# Autodesk Inventor assembly: ASY MSC Жабры
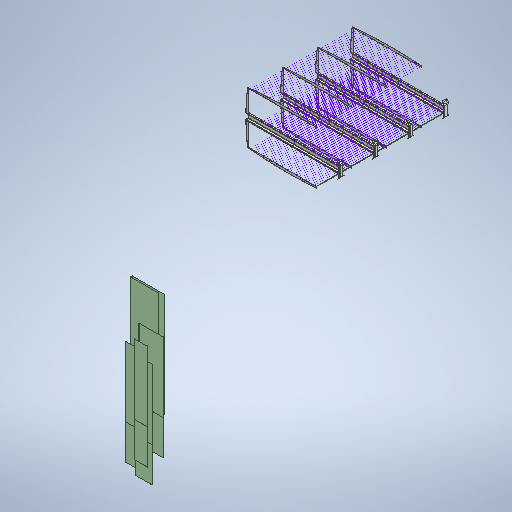
[picture p0: Inventor's stored thumbnail of the model, 512x512]
Saved by Autodesk Inventor 2025 (Build 290162010, 162A)
## iProperties
Created: 2024-08-31
Part Number: ASY MSC Жабры
Document SubType Name: Assembly
Designer: pokla
Author: pokla
## Documents named in this file (22)
- C:\Users\pokla\Documents\Inventor\Отстойник осветлитель\Manturovo_Se-clar-Gleb\ASY MSC Жабры.iam
- C:\Users\pokla\Documents\Inventor\Отстойник осветлитель\Manturovo_Se-clar-Gleb\MSC 0101 sheet gills.ipt
- C:\Users\pokla\Documents\Inventor\Отстойник осветлитель\Manturovo_Se-clar-Gleb\MSC 081 pillar 1.ipt
- C:\Users\pokla\Documents\Inventor\Отстойник осветлитель\Manturovo_Se-clar-Gleb\MSC 0102 sheet gills.ipt
- C:\Users\pokla\Documents\Inventor\Отстойник осветлитель\Manturovo_Se-clar-Gleb\MSC 0202 sheet gills.ipt
- C:\Users\pokla\Documents\Inventor\Отстойник осветлитель\Manturovo_Se-clar-Gleb\MSC 0103 sheet gills.ipt
- C:\Users\pokla\Documents\Inventor\Отстойник осветлитель\Manturovo_Se-clar-Gleb\MSC 0203 sheet gills.ipt
- C:\Users\pokla\Documents\Inventor\Отстойник осветлитель\Manturovo_Se-clar-Gleb\MSC 0104 sheet gills.ipt
- C:\Users\pokla\Documents\Inventor\Отстойник осветлитель\Manturovo_Se-clar-Gleb\MSC 0204 sheet gills.ipt
- C:\Users\pokla\Documents\Inventor\Отстойник осветлитель\Manturovo_Se-clar-Gleb\MSC 0105 sheet gills.ipt
- C:\Users\pokla\Documents\Inventor\Отстойник осветлитель\Manturovo_Se-clar-Gleb\MSC 0205 sheet gills.ipt
- C:\Users\pokla\Documents\Inventor\Отстойник осветлитель\Manturovo_Se-clar-Gleb\MSC 0106 sheet gills.ipt
- C:\Users\pokla\Documents\Inventor\Отстойник осветлитель\Manturovo_Se-clar-Gleb\MSC 0206 sheet gills.ipt
- C:\Users\pokla\Documents\Inventor\Отстойник осветлитель\Manturovo_Se-clar-Gleb\MSC 0107 sheet gills.ipt
- C:\Users\pokla\Documents\Inventor\Отстойник осветлитель\Manturovo_Se-clar-Gleb\MSC 0207 sheet gills.ipt
- C:\Users\pokla\Documents\Inventor\Отстойник осветлитель\Manturovo_Se-clar-Gleb\MSC 079 creen pillar.ipt
- C:\Users\pokla\Documents\Inventor\Отстойник осветлитель\Manturovo_Se-clar-Gleb\MSC DIM 085 tube belly.ipt
- C:\Users\pokla\Documents\Inventor\Отстойник осветлитель\Manturovo_Se-clar-Gleb\MSC 081 pillar 1_CPY.ipt
- C:\Users\pokla\Documents\Inventor\Отстойник осветлитель\Manturovo_Se-clar-Gleb\MSC 0211 string for sheets.ipt
- C:\Users\pokla\Documents\Inventor\Отстойник осветлитель\Manturovo_Se-clar-Gleb\MSC 079 top pillar.ipt
- C:\Users\pokla\Documents\Inventor\Отстойник осветлитель\Manturovo_Se-clar-Gleb\MSC DIM 085.1 heel.ipt
- C:\Users\pokla\Documents\Inventor\Отстойник осветлитель\Manturovo_Se-clar-Gleb\MSC 0201 sheet gills.ipt
## Components (184 placed, 21 different names)
1. MSC 0101 sheet gills.ipt:1 — Tangent:1, Tangent:2, Tangent:3, Flush:6, Flush:7, Flush:8, Mate:14
2. MSC 0201 sheet gills:1 — Flush:7, Flush:8, Mate:14
3. MSC 0102 sheet gills:1 — Rigid:17
4. MSC 0202 sheet gills:1 — Rigid:17
5. MSC 0103 sheet gills:1 — Rigid:18
6. MSC 0203 sheet gills:1 — Rigid:18
7. MSC 0104 sheet gills:1 — Rigid:19
8. MSC 0204 sheet gills:1 — Rigid:19
9. MSC 0105 sheet gills:1 — Rigid:20
10. MSC 0205 sheet gills:1 — Rigid:20
11. MSC 0106 sheet gills:1 — Rigid:21
12. MSC 0206 sheet gills:1 — Rigid:21
13. MSC 0107 sheet gills:1 — Rigid:22
14. MSC 0207 sheet gills:1 — Rigid:22
15. MSC 079 creen pillar:1 — Rigid:11, Rigid:12
16. MSC 081 pillar 1_CPY:1 — Rigid:8, Rigid:9
17. MSC 079 top pillar:1 — Rigid:8, Rigid:11
18. MSC 079 top pillar:2 — Rigid:9, Rigid:10
19. MSC 079 creen pillar:2 — Rigid:10, Rigid:15
20. MSC 081 pillar 1:1 — Mate:11, Mate:12, Mate:13, Rigid:13, Rigid:16, Flush:6
21. MSC DIM 085 tube belly:1 — Rigid:6, Rigid:7, Mate:11, Mate:12, Mate:13, Mate:15, Mate:16, Flush:9
22. MSC DIM 085.1 heel:1 — Rigid:7
23. MSC DIM 085.1 heel:2 — Rigid:6
24. MSC 079 creen pillar:3
25. MSC 081 pillar 1_CPY:2
26. MSC 079 top pillar:3
27. MSC 079 top pillar:4
28. MSC 079 creen pillar:4
29. MSC 081 pillar 1:2
30. MSC DIM 085 tube belly:2
31. MSC DIM 085.1 heel:3
32. MSC DIM 085.1 heel:4
33. MSC 079 creen pillar:5
34. MSC 081 pillar 1_CPY:3
35. MSC 079 top pillar:5
36. MSC 079 top pillar:6
37. MSC 079 creen pillar:6
38. MSC 081 pillar 1:3
39. MSC DIM 085 tube belly:3
40. MSC DIM 085.1 heel:5
41. MSC DIM 085.1 heel:6
42. MSC 079 creen pillar:7
43. MSC 081 pillar 1_CPY:4
44. MSC 079 top pillar:7
45. MSC 079 top pillar:8
46. MSC 079 creen pillar:8
47. MSC 081 pillar 1:4
48. MSC DIM 085 tube belly:4
49. MSC DIM 085.1 heel:7
50. MSC DIM 085.1 heel:8
51. MSC 0211 string for sheets:4 — Rigid:15
52. MSC 0211 string for sheets:2 — Rigid:12, Tangent:1, Tangent:2
53. MSC 0211 string for sheets:5
54. MSC 0211 string for sheets:6
55. MSC 0211 string for sheets:7
56. MSC 0211 string for sheets:8
57. MSC 0211 string for sheets:9
58. MSC 0211 string for sheets:10
59. MSC 0211 string for sheets:11
60. MSC 0211 string for sheets:12
61. MSC 0211 string for sheets:13
62. MSC 0211 string for sheets:14
63. MSC 0211 string for sheets:15
64. MSC 0211 string for sheets:16
65. MSC 0211 string for sheets:17
66. MSC 0211 string for sheets:18
67. MSC 0211 string for sheets:19
68. MSC 0211 string for sheets:20
69. MSC 0211 string for sheets:21
70. MSC 0211 string for sheets:22
71. MSC 0211 string for sheets:23
72. MSC 0211 string for sheets:24
73. MSC 0211 string for sheets:25
74. MSC 0211 string for sheets:26
75. MSC 0211 string for sheets:27
76. MSC 0211 string for sheets:28
77. MSC 0211 string for sheets:29
78. MSC 0211 string for sheets:30
79. MSC 0211 string for sheets:31
80. MSC 0211 string for sheets:32
81. MSC 0211 string for sheets:33
82. MSC 0211 string for sheets:34
83. MSC 0211 string for sheets:35
84. MSC 0211 string for sheets:36
85. MSC 0211 string for sheets:37
86. MSC 0211 string for sheets:38
87. MSC 0211 string for sheets:39
88. MSC 0211 string for sheets:40
89. MSC 0211 string for sheets:41
90. MSC 0211 string for sheets:42
91. MSC 0211 string for sheets:43
92. MSC 0211 string for sheets:44
93. MSC 0211 string for sheets:45
94. MSC 0211 string for sheets:46
95. MSC 0211 string for sheets:47
96. MSC 0211 string for sheets:48
97. MSC 0211 string for sheets:49
98. MSC 0211 string for sheets:50
99. MSC 0211 string for sheets:51
100. MSC 0211 string for sheets:52
101. MSC 0211 string for sheets:53
102. MSC 0211 string for sheets:54
103. MSC 0211 string for sheets:55
104. MSC 0211 string for sheets:56
105. MSC 0211 string for sheets:57
106. MSC 0211 string for sheets:58
107. MSC 0211 string for sheets:59
108. MSC 0211 string for sheets:60
109. MSC 0211 string for sheets:61
110. MSC 0211 string for sheets:62
111. MSC 0211 string for sheets:63
112. MSC 0211 string for sheets:64
113. MSC 0211 string for sheets:3 — Rigid:16
114. MSC 0211 string for sheets:1 — Rigid:13, Tangent:3
115. MSC 0211 string for sheets:65
116. MSC 0211 string for sheets:66
117. MSC 0211 string for sheets:67
118. MSC 0211 string for sheets:68
119. MSC 0211 string for sheets:69
120. MSC 0211 string for sheets:70
121. MSC 0211 string for sheets:71
122. MSC 0211 string for sheets:72
123. MSC 0211 string for sheets:73
124. MSC 0211 string for sheets:74
125. MSC 0211 string for sheets:75
126. MSC 0211 string for sheets:76
127. MSC 0211 string for sheets:77
128. MSC 0211 string for sheets:78
129. MSC 0211 string for sheets:79
130. MSC 0211 string for sheets:80
131. MSC 0211 string for sheets:81
132. MSC 0211 string for sheets:82
133. MSC 0211 string for sheets:83
134. MSC 0211 string for sheets:84
135. MSC 0211 string for sheets:85
136. MSC 0211 string for sheets:86
137. MSC 0211 string for sheets:87
138. MSC 0211 string for sheets:88
139. MSC 0211 string for sheets:89
140. MSC 0211 string for sheets:90
141. MSC 0211 string for sheets:91
142. MSC 0211 string for sheets:92
143. MSC 0211 string for sheets:93
144. MSC 0211 string for sheets:94
145. MSC 0211 string for sheets:95
146. MSC 0211 string for sheets:96
147. MSC 0211 string for sheets:97
148. MSC 0211 string for sheets:98
149. MSC 0211 string for sheets:99
150. MSC 0211 string for sheets:100
151. MSC 0211 string for sheets:101
152. MSC 0211 string for sheets:102
153. MSC 0211 string for sheets:103
154. MSC 0211 string for sheets:104
155. MSC 0211 string for sheets:105
156. MSC 0211 string for sheets:106
157. MSC 0211 string for sheets:107
158. MSC 0211 string for sheets:108
159. MSC 0211 string for sheets:109
160. MSC 0211 string for sheets:110
161. MSC 0211 string for sheets:111
162. MSC 0211 string for sheets:112
163. MSC 0211 string for sheets:113
164. MSC 0211 string for sheets:114
165. MSC 0211 string for sheets:115
166. MSC 0211 string for sheets:116
167. MSC 0211 string for sheets:117
168. MSC 0211 string for sheets:118
169. MSC 0211 string for sheets:119
170. MSC 0211 string for sheets:120
171. MSC 0211 string for sheets:121
172. MSC 0211 string for sheets:122
173. MSC 0211 string for sheets:123
174. MSC 0211 string for sheets:124
175. MSC 0211 string for sheets:125
176. MSC 0211 string for sheets:126
177. MSC 0211 string for sheets:127
178. MSC 0211 string for sheets:128
179. MSC 0211 string for sheets:129
180. MSC 0211 string for sheets:130
181. MSC 0211 string for sheets:131
182. MSC 0211 string for sheets:132
183. MSC 0211 string for sheets:133
184. MSC 0211 string for sheets:134
## Component patterns: (4 elements, first: MSC 079 creen pillar:1 + MSC 081 pillar 1_CPY:1 + MSC 079 top pillar:1 + MSC 079 top pillar:2 + MSC 079 creen pillar:2 + MSC 081 pillar 1:1 + MSC DIM 085 tube belly:1 + MSC DIM 085.1 heel:1 + MSC DIM 085.1 heel:2), (31 elements, first: MSC 0211 string for sheets:4 + MSC 0211 string for sheets:2), (36 elements, first: MSC 0211 string for sheets:3 + MSC 0211 string for sheets:1)
## Relationships (38: WeldJoint 17, Mate 12, Flush 6, Tangent 3)
- [Mate] (50 mm): MSC 0106 sheet gills:1 ↔ MSC 0107 sheet gills:1
- [Mate] (50 mm): MSC 0105 sheet gills:1 ↔ MSC 0106 sheet gills:1
- [Mate] (50 mm): MSC 0104 sheet gills:1 ↔ MSC 0105 sheet gills:1
- [Mate] (50 mm): MSC 0103 sheet gills:1 ↔ MSC 0104 sheet gills:1
- [Mate] (50 mm): MSC 0102 sheet gills:1 ↔ MSC 0103 sheet gills:1
- [Flush]: MSC 0102 sheet gills:1 ↔ MSC 0103 sheet gills:1
- [Flush]: MSC 0102 sheet gills:1 ↔ MSC 0103 sheet gills:1
- [WeldJoint]: MSC 081 pillar 1_CPY:1 ↔ MSC 081 pillar 1:1
- [Mate]: MSC 081 pillar 1_CPY:1 ↔ MSC 079 top pillar:1
- Rigid:6 [WeldJoint]: MSC DIM 085 tube belly:1 ↔ MSC DIM 085.1 heel:2
- Rigid:7 [WeldJoint]: MSC DIM 085 tube belly:1 ↔ MSC DIM 085.1 heel:1
- Mate:11: MSC 081 pillar 1:1 ↔ MSC DIM 085 tube belly:1
- Mate:12: MSC 081 pillar 1:1 ↔ MSC DIM 085 tube belly:1
- Mate:13: MSC 081 pillar 1:1 ↔ MSC DIM 085 tube belly:1
- Rigid:8 [WeldJoint]: MSC 081 pillar 1_CPY:1 ↔ MSC 079 top pillar:1
- Rigid:9 [WeldJoint]: MSC 081 pillar 1_CPY:1 ↔ MSC 079 top pillar:2
- Rigid:10 [WeldJoint]: MSC 079 top pillar:2 ↔ MSC 079 creen pillar:2
- Rigid:11 [WeldJoint]: MSC 079 creen pillar:1 ↔ MSC 079 top pillar:1
- Rigid:12 [WeldJoint] (-5 mm): MSC 079 creen pillar:1 ↔ MSC 0211 string for sheets:2
- Rigid:13 [WeldJoint] (-5 mm): MSC 081 pillar 1:1 ↔ MSC 0211 string for sheets:1
- Rigid:15 [WeldJoint] (-5 mm): MSC 079 creen pillar:2 ↔ MSC 0211 string for sheets:4
- Rigid:16 [WeldJoint] (-5 mm): MSC 081 pillar 1:1 ↔ MSC 0211 string for sheets:3
- Rigid:17 [WeldJoint]: MSC 0102 sheet gills:1 ↔ MSC 0202 sheet gills:1
- Rigid:18 [WeldJoint]: MSC 0103 sheet gills:1 ↔ MSC 0203 sheet gills:1
- Rigid:19 [WeldJoint]: MSC 0104 sheet gills:1 ↔ MSC 0204 sheet gills:1
- Rigid:20 [WeldJoint]: MSC 0105 sheet gills:1 ↔ MSC 0205 sheet gills:1
- Rigid:21 [WeldJoint]: MSC 0106 sheet gills:1 ↔ MSC 0206 sheet gills:1
- Rigid:22 [WeldJoint]: MSC 0107 sheet gills:1 ↔ MSC 0207 sheet gills:1
- Tangent:1: MSC 0101 sheet gills.ipt:1 ↔ MSC 0211 string for sheets:2
- Tangent:2: MSC 0101 sheet gills.ipt:1 ↔ MSC 0211 string for sheets:2
- Tangent:3: MSC 0101 sheet gills.ipt:1 ↔ MSC 0211 string for sheets:1
- Flush:6: MSC 0101 sheet gills.ipt:1 ↔ MSC 081 pillar 1:1
- Flush:7: MSC 0101 sheet gills.ipt:1 ↔ MSC 0201 sheet gills:1
- Flush:8: MSC 0101 sheet gills.ipt:1 ↔ MSC 0201 sheet gills:1
- Mate:14: MSC 0101 sheet gills.ipt:1 ↔ MSC 0201 sheet gills:1
- Mate:15: MSC DIM 085 tube belly:1
- Mate:16: MSC DIM 085 tube belly:1
- Flush:9: MSC DIM 085 tube belly:1
